# Autodesk Inventor assembly: #Spindexer
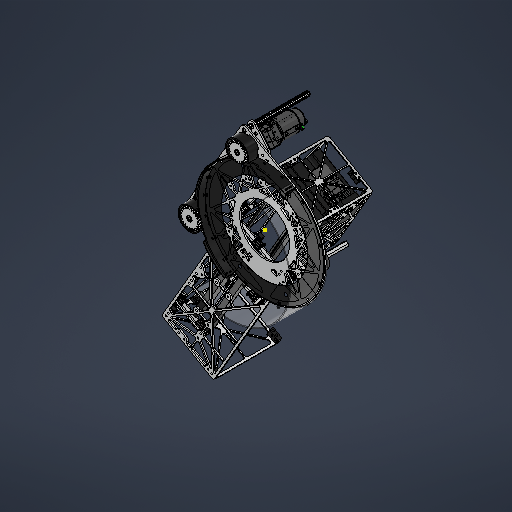
[picture p0: Inventor's stored thumbnail of the model, 512x512]
Saved by Autodesk Inventor 2026.1 (Build 301233020, 233B)
## iProperties
Created: 2026-02-05
Part Number: #Spindexer
Document SubType Name: Assembly
Designer: Owen L
Mass: 5573.01 g
Surface Area: 15044.5 cm^2
Volume: 3852.19 cm^3
Density: 1.44671 g/cm^3
Author: Owen L
## Documents named in this file (58)
- C:\Users\Owen\Documents\GitHub\2026-Robot-Mechanical\Spindexer\#Spindexer.iam
- C:\Users\Owen\Documents\GitHub\2026-Robot-Mechanical\Spindexer\3DPRINT,KICKER,RAMP.ipt
- C:\Users\Owen\Documents\GitHub\2026-Robot-Mechanical\#1_CAD Library\Power Transmission\Bearings\PURCHASED,HEX_BEARING.ipt
- C:\Users\Owen\Documents\GitHub\2026-Robot-Mechanical\#1_CAD Library\Building Materials\Fasteners\Nuts\PURCHASED,NYLOCK,10-32,NUT.ipt
- C:\Users\Owen\Documents\GitHub\2026-Robot-Mechanical\#1_CAD Library\Building Materials\Fasteners\Bolts\PURCHASED,10-32x0.625in,BUTTONHEAD,BOLT.ipt
- C:\Users\Owen\Documents\GitHub\2026-Robot-Mechanical\Spindexer\PLATE,SHOOTER,MOUNT.ipt
- C:\Users\Owen\Documents\GitHub\2026-Robot-Mechanical\Spindexer\PLATE,TURRET,ENCODER,GEAR.ipt
- C:\Users\Owen\Documents\GitHub\2026-Robot-Mechanical\Spindexer\PLATE,TURRET,PINNION,GEAR.ipt
- C:\Users\Owen\Documents\GitHub\2026-Robot-Mechanical\Spindexer\PLATE,TURRET,MOTOR,MOUNT.ipt
- C:\Users\Owen\Documents\GitHub\2026-Robot-Mechanical\#1_CAD Library\Electronics\CONTROLS,ENCODER,HEX_BORE.ipt
- C:\Users\Owen\Documents\GitHub\2026-Robot-Mechanical\Spindexer\STOCK,HEX,SHAFT,TURRET,DRIVE.ipt
- C:\Users\Owen\Documents\GitHub\2026-Robot-Mechanical\Spindexer\STOCK,HEX,SHAFT,TURRET,ENCODER.ipt
- C:\Users\Owen\Documents\GitHub\2026-Robot-Mechanical\Spindexer\3DPRINT,TURRET,HEX,SPACER.ipt
- C:\Users\Owen\Documents\GitHub\2026-Robot-Mechanical\Spindexer\STOCK,CHURRO,HEX,TURRET,MOTOR-MOUNT,SPACER.ipt
- C:\Users\Owen\Documents\GitHub\2026-Robot-Mechanical\#1_CAD Library\Building Materials\Fasteners\Bolts\PURCHASED,0.25-20x0.5in,BUTTONHEAD,BOLT.ipt
- C:\Users\Owen\Documents\GitHub\2026-Robot-Mechanical\Spindexer\MOTOR,VEX,FALCON,500.ipt
- C:\Users\Owen\Documents\GitHub\2026-Robot-Mechanical\#1_CAD Library\Power Transmission\MaxPlanetary\PURCHASED,REV,MAX-PLANETARY,SINGLE-STAGE,FALCON-TO-HEX.ipt
- C:\Users\Owen\Documents\GitHub\2026-Robot-Mechanical\#1_CAD Library\Building Materials\Fasteners\Washers\PURCHASED,WASHER,10-32.ipt
- C:\Users\Owen\Documents\GitHub\2026-Robot-Mechanical\Spindexer\3DPRINT,CABLE-SHROUD,QUARTER.ipt
- C:\Users\Owen\Documents\GitHub\2026-Robot-Mechanical\Spindexer\3DPRINT,CABLE,TRAY,BL.ipt
- C:\Users\Owen\Documents\GitHub\2026-Robot-Mechanical\Spindexer\3DPRINT,CABLE,TRAY,BR.ipt
- C:\Users\Owen\Documents\GitHub\2026-Robot-Mechanical\Spindexer\3DPRINT,CABLE,TRAY,TL.ipt
- C:\Users\Owen\Documents\GitHub\2026-Robot-Mechanical\Spindexer\3DPRINT,CABLE,TRAY,TR.ipt
- C:\Users\Owen\Documents\GitHub\2026-Robot-Mechanical\Spindexer\PLATE,SHOOTER,SHEILD,LOWER.ipt
- C:\Users\Owen\Documents\GitHub\2026-Robot-Mechanical\Spindexer\3DPRINT,TURRET,PINION,SHROUD.ipt
- C:\Users\Owen\Documents\GitHub\2026-Robot-Mechanical\#1_CAD Library\Building Materials\Fasteners\Bolts\PURCHASED,10-32x0.75in,BUTTONHEAD,BOLT.ipt
- C:\Users\Owen\Documents\GitHub\2026-Robot-Mechanical\Spindexer\3DPRINT,TURRET,PINION,SHROUD,21T.ipt
- C:\Users\Owen\Documents\GitHub\2026-Robot-Mechanical\Spindexer\STOCK,CHURRO,HEX,TURRET,MOTOR-MOUNT,SUPPORT.ipt
- C:\Users\Owen\Documents\GitHub\2026-Robot-Mechanical\Spindexer\PLATE,BACK.ipt
- C:\Users\Owen\Documents\GitHub\2026-Robot-Mechanical\Spindexer\PLATE,FRONT.ipt
- C:\Users\Owen\Documents\GitHub\2026-Robot-Mechanical\#1_CAD Library\Wheels\Compliant\PURCHASED,WHEEL,COMPLIANT,2.25in.ipt
- C:\Users\Owen\Documents\GitHub\2026-Robot-Mechanical\Spindexer\PLATE,BEARING,BLOCK.ipt
- C:\Users\Owen\Documents\GitHub\2026-Robot-Mechanical\Spindexer\PLATE,BEARING,BLOCK,TOP.ipt
- C:\Users\Owen\Documents\GitHub\2026-Robot-Mechanical\Spindexer\Kicker.ipt
- C:\Users\Owen\Documents\GitHub\2026-Robot-Mechanical\#1_CAD Library\Motors\MOTOR,NEO,V2.0.ipt
- C:\Users\Owen\Documents\GitHub\2026-Robot-Mechanical\Spindexer\PLATE_LEFT.ipt
- C:\Users\Owen\Documents\GitHub\2026-Robot-Mechanical\Spindexer\PLATE,BELT,REVERSER.ipt
- C:\Users\Owen\Documents\GitHub\2026-Robot-Mechanical\Spindexer\WCP-0562.ipt
- C:\Users\Owen\Documents\GitHub\2026-Robot-Mechanical\Spindexer\REV-21-1921.ipt
- C:\Users\Owen\Documents\GitHub\2026-Robot-Mechanical\Spindexer\WCP-2057.ipt
- C:\Users\Owen\Documents\GitHub\2026-Robot-Mechanical\Spindexer\WCP-1420.ipt
- C:\Users\Owen\Documents\GitHub\2026-Robot-Mechanical\Spindexer\STOCK,LEFT,HEX.ipt
- C:\Users\Owen\Documents\GitHub\2026-Robot-Mechanical\Spindexer\STOCK,REVERSER,HEX.ipt
- C:\Users\Owen\Documents\GitHub\2026-Robot-Mechanical\Spindexer\STOCK,TOP-RIGHT,HEX.ipt
- C:\Users\Owen\Documents\GitHub\2026-Robot-Mechanical\Spindexer\STOCK,BOTTOM-RIGHT,HEX.ipt
- C:\Users\Owen\Documents\GitHub\2026-Robot-Mechanical\Spindexer\3DPRINT,ROLLER,PLUG,SHORT.ipt
- C:\Users\Owen\Documents\GitHub\2026-Robot-Mechanical\Spindexer\3DPRINT,ROLLER,PLUG,LONG.ipt
- C:\Users\Owen\Documents\GitHub\2026-Robot-Mechanical\Spindexer\STOCK,KICKER,HEX.ipt
- C:\Users\Owen\Documents\GitHub\2026-Robot-Mechanical\Spindexer\3DPRINT,VERTICAL,ROLLER,TOP,BEARING,BLOCK.ipt
- C:\Users\Owen\Documents\GitHub\2026-Robot-Mechanical\Spindexer\WCP-0565.ipt
- C:\Users\Owen\Documents\GitHub\2026-Robot-Mechanical\Spindexer\3DPRINT,KICKER,MOTOR,MOUNT.ipt
- C:\Users\Owen\Documents\GitHub\2026-Robot-Mechanical\Spindexer\3DPRINT,NUT-BLOCK.ipt
- C:\Users\Owen\Documents\GitHub\2026-Robot-Mechanical\Spindexer\STOCK,REVERSER,STANDOFF.ipt
- C:\Users\Owen\Documents\GitHub\2026-Robot-Mechanical\Spindexer\3DPRINT,BELT,GUARD.ipt
- C:\Users\Owen\Documents\GitHub\2026-Robot-Mechanical\Spindexer\3DPRINT,BACK,RAIL.ipt
- C:\Users\Owen\Documents\GitHub\2026-Robot-Mechanical\Spindexer\PLATE,RIGHT.ipt
- C:\Users\Owen\Documents\GitHub\2026-Robot-Mechanical\Spindexer\STOCK,VERTICAL,HEX.ipt
- C:\Users\Owen\Documents\GitHub\2026-Robot-Mechanical\Spindexer\3DPRINT,LEFT,NUT-BLOCK.ipt
## Components (152 placed, 57 different names)
1. 3DPRINT,VERTICAL,ROLLER,TOP,BEARING,BLOCK:1 — Mate:309, Insert:317, Mate:359, Mate:360
2. 3DPRINT,TURRET,PINION,SHROUD:1 — Mate:224, Mate:225, Mate:226, Insert:267
3. PURCHASED,10-32x0.75in,BUTTONHEAD,BOLT:1 — Insert:268, Mate:232
4. PURCHASED,10-32x0.75in,BUTTONHEAD,BOLT:2 — Insert:267, Mate:236
5. 3DPRINT,TURRET,PINION,SHROUD,21T:1 — Mate:227, Mate:228, Mate:229, Insert:268
6. STOCK,CHURRO,HEX,TURRET,MOTOR-MOUNT,SPACER:7 — Insert:272
7. STOCK,CHURRO,HEX,TURRET,MOTOR-MOUNT,SPACER:8 — Insert:273
8. PURCHASED,0.25-20x0.5in,BUTTONHEAD,BOLT:16 — Insert:279
9. PURCHASED,0.25-20x0.5in,BUTTONHEAD,BOLT:17 — Insert:280
10. PURCHASED,0.25-20x0.5in,BUTTONHEAD,BOLT:18 — Insert:281
11. STOCK,CHURRO,HEX,TURRET,MOTOR-MOUNT,SUPPORT:1 — Insert:282
12. PLATE,BACK:1 — Mate:240, Mate:264, Flush:44, Flush:48, Flush:52, Mate:277, Mate:278, Mate:280, Insert:305, Insert:306, Insert:309, Insert:312, Insert:314, Insert:316, Mate:269, Insert:318, Mate:314, Mate:315, Insert:322, Insert:323, Mate:331, Mate:332, Insert:324, Insert:325, Mate:333, Mate:334, Mate:336, Mate:337, Mate:338, Insert:328, Insert:333, Insert:334, Insert:335, Insert:336, Insert:337, Insert:338, Mate:344, Insert:339, Mate:347, Flush:71, Mate:351, Flush:73, Mate:352, Flush:74, Flush:75, Mate:357, Flush:76, Insert:342, Mate:362
13. PLATE,FRONT:1 — Mate:264, Flush:44, Mate:265, Mate:268, Mate:270, Mate:274, Flush:51, Insert:311, Insert:313, Insert:315, Mate:306, Mate:311, Mate:323, Insert:320, Mate:325, Mate:327, Mate:328, Mate:329, Insert:326, Mate:335, Insert:327, Insert:331, Insert:332, Mate:339, Mate:340, Mate:343, Mate:345, Insert:340
14. PURCHASED,WHEEL,COMPLIANT,2.25in:1 — Mate:268, Mate:269, Insert:298, Mate:270
15. PURCHASED,WHEEL,COMPLIANT,2.25in:3 — Insert:298, Mate:309
16. PLATE,BEARING,BLOCK:1 — Flush:48, Flush:53, Insert:308
17. PLATE,BEARING,BLOCK,TOP:1 — Mate:272, Mate:278, Flush:53, Insert:310
18. KICKER_GEARBOX — Insert:304, Flush:50, Mate:323, Mate:325, Mate:326
19. MOTOR,NEO,V2.0:1 — Insert:304, Flush:50
20. PLATE,LEFT — Mate:274, Flush:51, Mate:275, Insert:341, Mate:353, Mate:354, Mate:355, Mate:356
21. PLATE,BELT,REVERSER:1 — Mate:280, Insert:307
22. WCP-0562:1 — Mate:285, Flush:56, Flush:58
23. REV-21-1921:1 — Mate:282, Flush:54
24. REV-21-1921:2 — Mate:281, Flush:54, Mate:290, Mate:291
25. WCP-2057:1 — Insert:308, Mate:287, Flush:59
26. WCP-2057:2 — Insert:307, Mate:283, Mate:291, Flush:60
27. WCP-2057:3 — Insert:306, Mate:282, Mate:287, Mate:292, Mate:296
28. WCP-2057:4 — Insert:305, Mate:281, Mate:288, Mate:289, Mate:297
29. WCP-2057:5 — Insert:311, Flush:62
30. WCP-2057:6 — Insert:310, Mate:286, Flush:61
31. WCP-2057:7 — Insert:313, Flush:63
32. WCP-2057:8 — Insert:309, Mate:284, Mate:285, Mate:286, Mate:295
33. WCP-2057:9 — Insert:312, Mate:293, Mate:299, Mate:316, Mate:318
34. WCP-2057:11 — Insert:314, Mate:294, Mate:300
35. WCP-2057:12 — Insert:316, Mate:319
36. WCP-2057:13 — Insert:315, Mate:301, Mate:302, Mate:305, Mate:324
37. WCP-1420:1 — Mate:283, Mate:288, Flush:55, Mate:289, Mate:290
38. WCP-1420:2 — Mate:284, Flush:55
39. WCP-0562:2 — Mate:292, Flush:56
40. WCP-0562:3 — Mate:293, Flush:57, Flush:58
41. WCP-0562:4 — Mate:294, Flush:57
42. STOCK,LEFT,HEX:1 — Mate:295, Flush:61
43. STOCK,LEFT,HEX:2 — Mate:296, Flush:59
44. STOCK,REVERSER,HEX:1 — Mate:297, Flush:60
45. STOCK,TOP-RIGHT,HEX:1 — Mate:299, Flush:62
46. STOCK,BOTTOM-RIGHT,HEX:1 — Mate:300, Flush:63
47. 3DPRINT,ROLLER,PLUG,SHORT:1
48. 3DPRINT,ROLLER,PLUG,LONG:1
49. STOCK,KICKER,HEX:1 — Mate:301
50. WCP-1420:3 — Mate:302, Flush:65, Mate:324
51. WCP-1420:5 — Mate:305, Mate:311
52. WCP-1420:6 — Mate:359, Mate:360, Flush:77
53. WCP-1420:7 — Mate:306, Flush:65, Mate:326
54. WCP-2057:14 — Insert:317, Mate:361
55. PLATE,BELT,REVERSER:2 — Mate:314, Mate:315, Insert:319
56. REV-21-1921:3 — Mate:317, Flush:66, Mate:321
57. WCP-2057:15 — Insert:318, Mate:317, Mate:320
58. REV-21-1921:4 — Mate:316, Mate:318, Flush:66
59. WCP-0565:1 — Mate:319, Flush:67
60. WCP-1420:8 — Mate:320, Mate:321, Mate:322, Flush:67
61. WCP-2057:16 — Insert:319, Mate:322
62. WCP-2057:17 — Insert:320
63. 3DPRINT,KICKER,MOTOR,MOUNT:1 — Mate:327, Mate:328, Mate:329
64. 3DPRINT,NUT-BLOCK:1 — Insert:321, Mate:330
65. 3DPRINT,NUT-BLOCK:2 — Insert:323, Mate:332
66. 3DPRINT,NUT-BLOCK:3 — Insert:322, Mate:331
67. 3DPRINT,NUT-BLOCK:4 — Insert:324, Mate:333
68. 3DPRINT,NUT-BLOCK:5 — Insert:325, Mate:334
69. 3DPRINT,NUT-BLOCK:6 — Insert:326, Mate:335
70. 3DPRINT,NUT-BLOCK:7 — Mate:336, Mate:337, Mate:338
71. 3DPRINT,NUT-BLOCK:8 — Insert:327, Mate:343
72. 3DPRINT,NUT-BLOCK:9 — Insert:332, Mate:339
73. 3DPRINT,NUT-BLOCK:10 — Insert:331, Mate:340
74. 3DPRINT,NUT-BLOCK:11 — Mate:345, Insert:340
75. 3DPRINT,NUT-BLOCK:12 — Mate:344, Insert:339
76. 3DPRINT,NUT-BLOCK:13 — Insert:328
77. STOCK,REVERSER,STANDOFF:1 — Insert:333
78. STOCK,REVERSER,STANDOFF:2 — Insert:334
79. STOCK,REVERSER,STANDOFF:3 — Insert:335
80. STOCK,REVERSER,STANDOFF:4 — Insert:338
81. STOCK,REVERSER,STANDOFF:5 — Insert:337
82. STOCK,REVERSER,STANDOFF:6 — Insert:336
83. 3DPRINT,BELT,GUARD:1 — Mate:346, Mate:347, Mate:348, Flush:68, Flush:72
84. 3DPRINT,BELT,GUARD:2 — Mate:348, Mate:349, Flush:68
85. 3DPRINT,BELT,GUARD:3 — Flush:70, Flush:71, Mate:351, Flush:72
86. 3DPRINT,BELT,GUARD:4 — Flush:70, Flush:73
87. 3DPRINT,BACK,RAIL:1 — Mate:352, Flush:74, Flush:75
88. 3DPRINT,NUT-BLOCK:14 — Insert:341, Mate:353
89. 3DPRINT,NUT-BLOCK:15 — Mate:354, Mate:355, Mate:356
90. PLATE,RIGHT:1 — Mate:357, Mate:358, Flush:76, Mate:364, Insert:344
91. STOCK,VERTICAL,HEX:1 — Mate:361, Flush:77
92. 3DPRINT,NUT-BLOCK:16 — Insert:343, Mate:363
93. 3DPRINT,NUT-BLOCK:17 — Insert:342, Mate:362
94. 3DPRINT,LEFT,NUT-BLOCK:1 — Mate:364, Insert:344
95. PURCHASED,10-32x0.625in,BUTTONHEAD,BOLT:45 — Insert:233
96. PURCHASED,NYLOCK,10-32,NUT:5 — Insert:234
97. PURCHASED,NYLOCK,10-32,NUT:6 — Insert:232
98. PURCHASED,0.25-20x0.5in,BUTTONHEAD,BOLT:9 — Insert:163
99. PURCHASED,0.25-20x0.5in,BUTTONHEAD,BOLT:8 — Insert:162
100. PURCHASED,0.25-20x0.5in,BUTTONHEAD,BOLT:6 — Insert:159
101. PURCHASED,0.25-20x0.5in,BUTTONHEAD,BOLT:5 — Insert:270
102. PURCHASED,NYLOCK,10-32,NUT:8 — Insert:236
103. PURCHASED,NYLOCK,10-32,NUT:7 — Insert:238
104. PURCHASED,10-32x0.625in,BUTTONHEAD,BOLT:47 — Insert:235
105. PURCHASED,0.25-20x0.5in,BUTTONHEAD,BOLT:4 — Insert:158
106. PURCHASED,10-32x0.625in,BUTTONHEAD,BOLT:61 — Insert:174
107. PURCHASED,10-32x0.625in,BUTTONHEAD,BOLT:60 — Insert:175
108. PURCHASED,10-32x0.625in,BUTTONHEAD,BOLT:59 — Insert:176
109. PURCHASED,10-32x0.625in,BUTTONHEAD,BOLT:58 — Insert:177
110. PURCHASED,0.25-20x0.5in,BUTTONHEAD,BOLT:15 — Insert:277
111. PURCHASED,0.25-20x0.5in,BUTTONHEAD,BOLT:14 — Insert:278
112. PURCHASED,0.25-20x0.5in,BUTTONHEAD,BOLT:13
113. PURCHASED,0.25-20x0.5in,BUTTONHEAD,BOLT:12 — Insert:276
114. PURCHASED,0.25-20x0.5in,BUTTONHEAD,BOLT:11 — Insert:169
115. PURCHASED,0.25-20x0.5in,BUTTONHEAD,BOLT:10 — Insert:168
116. PURCHASED,WASHER,10-32:11 — Insert:215, Insert:218
117. PURCHASED,WASHER,10-32:12 — Insert:217, Insert:220
118. PURCHASED,WASHER,10-32:13 — Insert:216, Insert:219
119. PURCHASED,10-32x0.625in,BUTTONHEAD,BOLT:62 — Insert:218
120. PURCHASED,10-32x0.625in,BUTTONHEAD,BOLT:63 — Insert:219
121. PURCHASED,10-32x0.625in,BUTTONHEAD,BOLT:64 — Insert:220
122. 3DPRINT,TURRET,HEX,SPACER:1 — Mate:94, Mate:102, Mate:144, Mate:145
123. 3DPRINT,TURRET,HEX,SPACER:2 — Mate:93, Mate:141, Mate:142
124. 3DPRINT,KICKER,RAMP:1 — Flush:52, Mate:277
125. 3DPRINT,CABLE,TRAY,TR:1 — Mate:219, Mate:220
126. 3DPRINT,CABLE,TRAY,TL:1 — Mate:217, Mate:218, Mate:219, Mate:220
127. 3DPRINT,CABLE,TRAY,BR:1 — Mate:215, Mate:216, Mate:217, Mate:218
128. 3DPRINT,CABLE,TRAY,BL:1 — Mate:213, Mate:214, Flush:33, Mate:215, Mate:216
129. 3DPRINT,CABLE-SHROUD,QUARTER:2 — Mate:205, Mate:206, Mate:207, Mate:223, Mate:226
130. 3DPRINT,CABLE-SHROUD,QUARTER:1 — Mate:202, Mate:203, Mate:204, Mate:205, Mate:207, Flush:33, Mate:228
131. PLATE,SHOOTER,MOUNT:1 — Mate:82, Mate:95, Mate:100, Insert:150, Insert:152, Insert:153, Insert:154, Insert:158, Insert:159, Insert:165, Insert:166, Insert:168, Insert:169, Insert:233, Insert:235, Mate:202, Mate:203, Mate:204, Mate:206, Mate:213, Mate:214, Mate:222, Flush:34, Mate:225, Mate:229, Mate:231, Insert:270, Mate:233, Mate:234, Mate:235, Insert:274, Insert:276, Insert:280, Insert:281, Mate:240, Mate:265, Mate:272, Mate:275, Insert:321, Mate:330, Mate:346, Mate:349, Mate:358, Insert:343, Mate:363
132. PLATE,TURRET,MOTOR,MOUNT:1 — Mate:100, Insert:155, Insert:157, Insert:162, Insert:163, Insert:174, Insert:175, Insert:176, Insert:177, Mate:147, Insert:178, Mate:148, Mate:231, Insert:269, Insert:282
133. PLATE,TURRET,MOTOR,MOUNT:2 — Mate:233, Mate:234, Mate:235, Insert:271, Insert:272, Insert:273, Insert:275, Insert:277, Insert:278, Insert:279
134. PLATE,TURRET,ENCODER,GEAR:1 — Mate:102, Mate:143, Flush:26
135. PLATE,TURRET,PINNION,GEAR:1 — Mate:86, Flush:25, Mate:140, Mate:141
136. PLATE,SHOOTER,SHEILD,LOWER:1 — Mate:222, Flush:34, Mate:223
137. STOCK,CHURRO,HEX,TURRET,MOTOR-MOUNT,SPACER:5 — Insert:165
138. STOCK,CHURRO,HEX,TURRET,MOTOR-MOUNT,SPACER:6 — Insert:166
139. STOCK,CHURRO,HEX,TURRET,MOTOR-MOUNT,SPACER:4 — Insert:271, Insert:274
140. STOCK,CHURRO,HEX,TURRET,MOTOR-MOUNT,SPACER:3 — Insert:269
141. STOCK,CHURRO,HEX,TURRET,MOTOR-MOUNT,SPACER:2 — Insert:152, Insert:157
142. STOCK,CHURRO,HEX,TURRET,MOTOR-MOUNT,SPACER:1 — Insert:150
143. STOCK,HEX,SHAFT,TURRET,ENCODER:1 — Mate:143, Flush:26, Mate:144, Insert:216, Insert:217, Mate:224
144. STOCK,HEX,SHAFT,TURRET,DRIVE:1 — Flush:25, Mate:140, Mate:142, Insert:215, Mate:227
145. PURCHASED,HEX_BEARING:6 — Mate:83, Mate:86, Mate:93, Insert:154
146. PURCHASED,HEX_BEARING:7 — Mate:94, Mate:96, Insert:153, Mate:145
147. CONTROLS,ENCODER,HEX_BORE:1 — Mate:95, Mate:96, Insert:236, Insert:238, Mate:236
148. CONTROLS,ENCODER,HEX_BORE:2 — Mate:82, Mate:83, Insert:232, Insert:234, Mate:232
149. PURCHASED,HEX_BEARING:8 — Insert:155
150. MOTOR,VEX,FALCON,500:1 — Insert:179, Mate:149
151. PURCHASED,REV,MAX-PLANETARY,SINGLE-STAGE,FALCON-TO-HEX:1 — Mate:147, Insert:178, Mate:148, Insert:179, Mate:149
152. PURCHASED,HEX_BEARING:9 — Insert:275
## Relationships (256: Mate 135, Insert 88, Flush 33)
- Mate:82: PLATE,SHOOTER,MOUNT:1 ↔ CONTROLS,ENCODER,HEX_BORE:2
- Mate:83: PURCHASED,HEX_BEARING:6 ↔ CONTROLS,ENCODER,HEX_BORE:2
- Mate:86: PLATE,TURRET,PINNION,GEAR:1 ↔ PURCHASED,HEX_BEARING:6
- Mate:93: 3DPRINT,TURRET,HEX,SPACER:2 ↔ PURCHASED,HEX_BEARING:6
- Mate:94: 3DPRINT,TURRET,HEX,SPACER:1 ↔ PURCHASED,HEX_BEARING:7
- Mate:95: PLATE,SHOOTER,MOUNT:1 ↔ CONTROLS,ENCODER,HEX_BORE:1
- Mate:96: PURCHASED,HEX_BEARING:7 ↔ CONTROLS,ENCODER,HEX_BORE:1
- Mate:100 (19.05 mm): PLATE,SHOOTER,MOUNT:1 ↔ PLATE,TURRET,MOTOR,MOUNT:1
- Mate:102: 3DPRINT,TURRET,HEX,SPACER:1 ↔ PLATE,TURRET,ENCODER,GEAR:1
- Insert:150: PLATE,SHOOTER,MOUNT:1 ↔ STOCK,CHURRO,HEX,TURRET,MOTOR-MOUNT,SPACER:1
- Insert:152: PLATE,SHOOTER,MOUNT:1 ↔ STOCK,CHURRO,HEX,TURRET,MOTOR-MOUNT,SPACER:2
- Insert:153: PLATE,SHOOTER,MOUNT:1 ↔ PURCHASED,HEX_BEARING:7
- Insert:154: PLATE,SHOOTER,MOUNT:1 ↔ PURCHASED,HEX_BEARING:6
- Insert:155: PLATE,TURRET,MOTOR,MOUNT:1 ↔ PURCHASED,HEX_BEARING:8
- Insert:157: PLATE,TURRET,MOTOR,MOUNT:1 ↔ STOCK,CHURRO,HEX,TURRET,MOTOR-MOUNT,SPACER:2
- Insert:158: PURCHASED,0.25-20x0.5in,BUTTONHEAD,BOLT:4 ↔ PLATE,SHOOTER,MOUNT:1
- Insert:159: PURCHASED,0.25-20x0.5in,BUTTONHEAD,BOLT:6 ↔ PLATE,SHOOTER,MOUNT:1
- Insert:162: PURCHASED,0.25-20x0.5in,BUTTONHEAD,BOLT:8 ↔ PLATE,TURRET,MOTOR,MOUNT:1
- Insert:163: PURCHASED,0.25-20x0.5in,BUTTONHEAD,BOLT:9 ↔ PLATE,TURRET,MOTOR,MOUNT:1
- Flush:25: PLATE,TURRET,PINNION,GEAR:1 ↔ STOCK,HEX,SHAFT,TURRET,DRIVE:1
- Mate:140: PLATE,TURRET,PINNION,GEAR:1 ↔ STOCK,HEX,SHAFT,TURRET,DRIVE:1
- Mate:141: 3DPRINT,TURRET,HEX,SPACER:2 ↔ PLATE,TURRET,PINNION,GEAR:1
- Mate:142: 3DPRINT,TURRET,HEX,SPACER:2 ↔ STOCK,HEX,SHAFT,TURRET,DRIVE:1
- Mate:143: PLATE,TURRET,ENCODER,GEAR:1 ↔ STOCK,HEX,SHAFT,TURRET,ENCODER:1
- Flush:26: PLATE,TURRET,ENCODER,GEAR:1 ↔ STOCK,HEX,SHAFT,TURRET,ENCODER:1
- Mate:144: 3DPRINT,TURRET,HEX,SPACER:1 ↔ STOCK,HEX,SHAFT,TURRET,ENCODER:1
- Mate:145: 3DPRINT,TURRET,HEX,SPACER:1 ↔ PURCHASED,HEX_BEARING:7
- Insert:165: PLATE,SHOOTER,MOUNT:1 ↔ STOCK,CHURRO,HEX,TURRET,MOTOR-MOUNT,SPACER:5
- Insert:166: PLATE,SHOOTER,MOUNT:1 ↔ STOCK,CHURRO,HEX,TURRET,MOTOR-MOUNT,SPACER:6
- Insert:168: PURCHASED,0.25-20x0.5in,BUTTONHEAD,BOLT:10 ↔ PLATE,SHOOTER,MOUNT:1
- Insert:169: PURCHASED,0.25-20x0.5in,BUTTONHEAD,BOLT:11 ↔ PLATE,SHOOTER,MOUNT:1
- Insert:174: PURCHASED,10-32x0.625in,BUTTONHEAD,BOLT:61 ↔ PLATE,TURRET,MOTOR,MOUNT:1
- Insert:175: PURCHASED,10-32x0.625in,BUTTONHEAD,BOLT:60 ↔ PLATE,TURRET,MOTOR,MOUNT:1
- Insert:176: PURCHASED,10-32x0.625in,BUTTONHEAD,BOLT:59 ↔ PLATE,TURRET,MOTOR,MOUNT:1
- Insert:177: PURCHASED,10-32x0.625in,BUTTONHEAD,BOLT:58 ↔ PLATE,TURRET,MOTOR,MOUNT:1
- Mate:147: PLATE,TURRET,MOTOR,MOUNT:1 ↔ PURCHASED,REV,MAX-PLANETARY,SINGLE-STAGE,FALCON-TO-HEX:1
- Insert:178: PLATE,TURRET,MOTOR,MOUNT:1 ↔ PURCHASED,REV,MAX-PLANETARY,SINGLE-STAGE,FALCON-TO-HEX:1
- Mate:148: PLATE,TURRET,MOTOR,MOUNT:1 ↔ PURCHASED,REV,MAX-PLANETARY,SINGLE-STAGE,FALCON-TO-HEX:1
- Insert:179: MOTOR,VEX,FALCON,500:1 ↔ PURCHASED,REV,MAX-PLANETARY,SINGLE-STAGE,FALCON-TO-HEX:1
- Mate:149: MOTOR,VEX,FALCON,500:1 ↔ PURCHASED,REV,MAX-PLANETARY,SINGLE-STAGE,FALCON-TO-HEX:1
- Insert:215: PURCHASED,WASHER,10-32:11 ↔ STOCK,HEX,SHAFT,TURRET,DRIVE:1
- Insert:216: PURCHASED,WASHER,10-32:13 ↔ STOCK,HEX,SHAFT,TURRET,ENCODER:1
- Insert:217: PURCHASED,WASHER,10-32:12 ↔ STOCK,HEX,SHAFT,TURRET,ENCODER:1
- Insert:218: PURCHASED,WASHER,10-32:11 ↔ PURCHASED,10-32x0.625in,BUTTONHEAD,BOLT:62
- Insert:219: PURCHASED,WASHER,10-32:13 ↔ PURCHASED,10-32x0.625in,BUTTONHEAD,BOLT:63
- Insert:220: PURCHASED,WASHER,10-32:12 ↔ PURCHASED,10-32x0.625in,BUTTONHEAD,BOLT:64
- Insert:232: PURCHASED,NYLOCK,10-32,NUT:6 ↔ CONTROLS,ENCODER,HEX_BORE:2
- Insert:233: PURCHASED,10-32x0.625in,BUTTONHEAD,BOLT:45 ↔ PLATE,SHOOTER,MOUNT:1
- Insert:234: PURCHASED,NYLOCK,10-32,NUT:5 ↔ CONTROLS,ENCODER,HEX_BORE:2
- Insert:235: PURCHASED,10-32x0.625in,BUTTONHEAD,BOLT:47 ↔ PLATE,SHOOTER,MOUNT:1
- Insert:236: PURCHASED,NYLOCK,10-32,NUT:8 ↔ CONTROLS,ENCODER,HEX_BORE:1
- Insert:238: PURCHASED,NYLOCK,10-32,NUT:7 ↔ CONTROLS,ENCODER,HEX_BORE:1
- Mate:202: 3DPRINT,CABLE-SHROUD,QUARTER:1 ↔ PLATE,SHOOTER,MOUNT:1
- Mate:203: 3DPRINT,CABLE-SHROUD,QUARTER:1 ↔ PLATE,SHOOTER,MOUNT:1
- Mate:204: 3DPRINT,CABLE-SHROUD,QUARTER:1 ↔ PLATE,SHOOTER,MOUNT:1
- Mate:205: 3DPRINT,CABLE-SHROUD,QUARTER:2 ↔ 3DPRINT,CABLE-SHROUD,QUARTER:1
- Mate:206: 3DPRINT,CABLE-SHROUD,QUARTER:2 ↔ PLATE,SHOOTER,MOUNT:1
- Mate:207: 3DPRINT,CABLE-SHROUD,QUARTER:2 ↔ 3DPRINT,CABLE-SHROUD,QUARTER:1
- Mate:213: 3DPRINT,CABLE,TRAY,BL:1 ↔ PLATE,SHOOTER,MOUNT:1
- Mate:214: 3DPRINT,CABLE,TRAY,BL:1 ↔ PLATE,SHOOTER,MOUNT:1
- Flush:33: 3DPRINT,CABLE,TRAY,BL:1 ↔ 3DPRINT,CABLE-SHROUD,QUARTER:1
- Mate:215: 3DPRINT,CABLE,TRAY,BR:1 ↔ 3DPRINT,CABLE,TRAY,BL:1
- Mate:216: 3DPRINT,CABLE,TRAY,BR:1 ↔ 3DPRINT,CABLE,TRAY,BL:1
- Mate:217: 3DPRINT,CABLE,TRAY,TL:1 ↔ 3DPRINT,CABLE,TRAY,BR:1
- Mate:218: 3DPRINT,CABLE,TRAY,TL:1 ↔ 3DPRINT,CABLE,TRAY,BR:1
- Mate:219: 3DPRINT,CABLE,TRAY,TR:1 ↔ 3DPRINT,CABLE,TRAY,TL:1
- Mate:220: 3DPRINT,CABLE,TRAY,TR:1 ↔ 3DPRINT,CABLE,TRAY,TL:1
- Mate:222: PLATE,SHOOTER,MOUNT:1 ↔ PLATE,SHOOTER,SHEILD,LOWER:1
- Flush:34: PLATE,SHOOTER,MOUNT:1 ↔ PLATE,SHOOTER,SHEILD,LOWER:1
- Mate:223: 3DPRINT,CABLE-SHROUD,QUARTER:2 ↔ PLATE,SHOOTER,SHEILD,LOWER:1
- Mate:224: 3DPRINT,TURRET,PINION,SHROUD:1 ↔ STOCK,HEX,SHAFT,TURRET,ENCODER:1
- Mate:225: 3DPRINT,TURRET,PINION,SHROUD:1 ↔ PLATE,SHOOTER,MOUNT:1
- Mate:226: 3DPRINT,TURRET,PINION,SHROUD:1 ↔ 3DPRINT,CABLE-SHROUD,QUARTER:2
- Insert:267: 3DPRINT,TURRET,PINION,SHROUD:1 ↔ PURCHASED,10-32x0.75in,BUTTONHEAD,BOLT:2
- Mate:227: 3DPRINT,TURRET,PINION,SHROUD,21T:1 ↔ STOCK,HEX,SHAFT,TURRET,DRIVE:1
- Mate:228: 3DPRINT,TURRET,PINION,SHROUD,21T:1 ↔ 3DPRINT,CABLE-SHROUD,QUARTER:1
- Mate:229: 3DPRINT,TURRET,PINION,SHROUD,21T:1 ↔ PLATE,SHOOTER,MOUNT:1
- Insert:268: PURCHASED,10-32x0.75in,BUTTONHEAD,BOLT:1 ↔ 3DPRINT,TURRET,PINION,SHROUD,21T:1
- Mate:231: PLATE,SHOOTER,MOUNT:1 ↔ PLATE,TURRET,MOTOR,MOUNT:1
- Insert:269: PLATE,TURRET,MOTOR,MOUNT:1 ↔ STOCK,CHURRO,HEX,TURRET,MOTOR-MOUNT,SPACER:3
- Insert:270: PURCHASED,0.25-20x0.5in,BUTTONHEAD,BOLT:5 ↔ PLATE,SHOOTER,MOUNT:1
- Mate:232: PURCHASED,10-32x0.75in,BUTTONHEAD,BOLT:1 ↔ CONTROLS,ENCODER,HEX_BORE:2
- Mate:233: PLATE,SHOOTER,MOUNT:1 ↔ PLATE,TURRET,MOTOR,MOUNT:2
- Mate:234: PLATE,SHOOTER,MOUNT:1 ↔ PLATE,TURRET,MOTOR,MOUNT:2
- Mate:235: PLATE,SHOOTER,MOUNT:1 ↔ PLATE,TURRET,MOTOR,MOUNT:2
- Insert:271: PLATE,TURRET,MOTOR,MOUNT:2 ↔ STOCK,CHURRO,HEX,TURRET,MOTOR-MOUNT,SPACER:4
- Insert:272: STOCK,CHURRO,HEX,TURRET,MOTOR-MOUNT,SPACER:7 ↔ PLATE,TURRET,MOTOR,MOUNT:2
- Insert:273: STOCK,CHURRO,HEX,TURRET,MOTOR-MOUNT,SPACER:8 ↔ PLATE,TURRET,MOTOR,MOUNT:2
- Insert:274: PLATE,SHOOTER,MOUNT:1 ↔ STOCK,CHURRO,HEX,TURRET,MOTOR-MOUNT,SPACER:4
- Insert:275: PLATE,TURRET,MOTOR,MOUNT:2 ↔ PURCHASED,HEX_BEARING:9
- Insert:276: PURCHASED,0.25-20x0.5in,BUTTONHEAD,BOLT:12 ↔ PLATE,SHOOTER,MOUNT:1
- Insert:277: PURCHASED,0.25-20x0.5in,BUTTONHEAD,BOLT:15 ↔ PLATE,TURRET,MOTOR,MOUNT:2
- Insert:278: PURCHASED,0.25-20x0.5in,BUTTONHEAD,BOLT:14 ↔ PLATE,TURRET,MOTOR,MOUNT:2
- Mate:236: PURCHASED,10-32x0.75in,BUTTONHEAD,BOLT:2 ↔ CONTROLS,ENCODER,HEX_BORE:1
- Insert:279: PURCHASED,0.25-20x0.5in,BUTTONHEAD,BOLT:16 ↔ PLATE,TURRET,MOTOR,MOUNT:2
- Insert:280: PURCHASED,0.25-20x0.5in,BUTTONHEAD,BOLT:17 ↔ PLATE,SHOOTER,MOUNT:1
- Insert:281: PURCHASED,0.25-20x0.5in,BUTTONHEAD,BOLT:18 ↔ PLATE,SHOOTER,MOUNT:1
- Insert:282: STOCK,CHURRO,HEX,TURRET,MOTOR-MOUNT,SUPPORT:1 ↔ PLATE,TURRET,MOTOR,MOUNT:1
- Mate:240: PLATE,BACK:1 ↔ PLATE,SHOOTER,MOUNT:1
- Mate:264 (158.75 mm): PLATE,BACK:1 ↔ PLATE,FRONT:1
- Flush:44: PLATE,BACK:1 ↔ PLATE,FRONT:1
- Mate:265: PLATE,FRONT:1 ↔ PLATE,SHOOTER,MOUNT:1
- Mate:268 (-208.788 mm): PLATE,FRONT:1 ↔ PURCHASED,WHEEL,COMPLIANT,2.25in:1
- Mate:269 (179.832 mm): PLATE,BACK:1 ↔ PURCHASED,WHEEL,COMPLIANT,2.25in:1
- Insert:298: PURCHASED,WHEEL,COMPLIANT,2.25in:1 ↔ PURCHASED,WHEEL,COMPLIANT,2.25in:3
- Mate:270 (6.35 mm): PLATE,FRONT:1 ↔ PURCHASED,WHEEL,COMPLIANT,2.25in:1
- Mate:272: PLATE,BEARING,BLOCK,TOP:1 ↔ PLATE,SHOOTER,MOUNT:1
- Flush:48: PLATE,BACK:1 ↔ PLATE,BEARING,BLOCK:1
- Insert:304: KICKER_GEARBOX ↔ MOTOR,NEO,V2.0:1
- Flush:50: KICKER_GEARBOX ↔ MOTOR,NEO,V2.0:1
- Mate:274: PLATE,FRONT:1 ↔ PLATE,LEFT
- Flush:51: PLATE,FRONT:1 ↔ PLATE,LEFT
- Mate:275: PLATE,LEFT ↔ PLATE,SHOOTER,MOUNT:1
- Flush:52: PLATE,BACK:1 ↔ 3DPRINT,KICKER,RAMP:1
- Mate:277: PLATE,BACK:1 ↔ 3DPRINT,KICKER,RAMP:1
- Mate:278 (95.25 mm): PLATE,BACK:1 ↔ PLATE,BEARING,BLOCK,TOP:1
- Flush:53: PLATE,BEARING,BLOCK:1 ↔ PLATE,BEARING,BLOCK,TOP:1
- Mate:280: PLATE,BACK:1 ↔ PLATE,BELT,REVERSER:1
- Insert:305: PLATE,BACK:1 ↔ WCP-2057:4
- Insert:306: PLATE,BACK:1 ↔ WCP-2057:3
- Insert:307: PLATE,BELT,REVERSER:1 ↔ WCP-2057:2
- Insert:308: PLATE,BEARING,BLOCK:1 ↔ WCP-2057:1
- Insert:309: PLATE,BACK:1 ↔ WCP-2057:8
- Insert:310: PLATE,BEARING,BLOCK,TOP:1 ↔ WCP-2057:6
- Insert:311: PLATE,FRONT:1 ↔ WCP-2057:5
- Insert:312: PLATE,BACK:1 ↔ WCP-2057:9
- Insert:313: PLATE,FRONT:1 ↔ WCP-2057:7
- Insert:314: PLATE,BACK:1 ↔ WCP-2057:11
- Insert:315: PLATE,FRONT:1 ↔ WCP-2057:13
- Insert:316: PLATE,BACK:1 ↔ WCP-2057:12
- Mate:281: REV-21-1921:2 ↔ WCP-2057:4
- Mate:282: REV-21-1921:1 ↔ WCP-2057:3
- Flush:54: REV-21-1921:1 ↔ REV-21-1921:2
- Mate:283: WCP-2057:2 ↔ WCP-1420:1
- Mate:284: WCP-2057:8 ↔ WCP-1420:2
- Mate:285: WCP-0562:1 ↔ WCP-2057:8
- Mate:286: WCP-2057:6 ↔ WCP-2057:8
- Mate:287: WCP-2057:1 ↔ WCP-2057:3
- Mate:288: WCP-2057:4 ↔ WCP-1420:1
- Flush:55: WCP-1420:1 ↔ WCP-1420:2
- Mate:289: WCP-2057:4 ↔ WCP-1420:1
- Mate:290: REV-21-1921:2 ↔ WCP-1420:1
- Mate:291: REV-21-1921:2 ↔ WCP-2057:2
- Mate:292: WCP-2057:3 ↔ WCP-0562:2
- Mate:293: WCP-2057:9 ↔ WCP-0562:3
- Mate:294: WCP-2057:11 ↔ WCP-0562:4
- Flush:56: WCP-0562:1 ↔ WCP-0562:2
- Flush:57: WCP-0562:3 ↔ WCP-0562:4
- Flush:58: WCP-0562:1 ↔ WCP-0562:3
- Mate:295: WCP-2057:8 ↔ STOCK,LEFT,HEX:1
- Mate:296: WCP-2057:3 ↔ STOCK,LEFT,HEX:2
- Mate:297: WCP-2057:4 ↔ STOCK,REVERSER,HEX:1
- Mate:299: WCP-2057:9 ↔ STOCK,TOP-RIGHT,HEX:1
- Mate:300: WCP-2057:11 ↔ STOCK,BOTTOM-RIGHT,HEX:1
- Flush:59: WCP-2057:1 ↔ STOCK,LEFT,HEX:2
- Flush:60: WCP-2057:2 ↔ STOCK,REVERSER,HEX:1
- Flush:61: WCP-2057:6 ↔ STOCK,LEFT,HEX:1
- Flush:62: WCP-2057:5 ↔ STOCK,TOP-RIGHT,HEX:1
- Flush:63: WCP-2057:7 ↔ STOCK,BOTTOM-RIGHT,HEX:1
- Mate:301: WCP-2057:13 ↔ STOCK,KICKER,HEX:1
- Mate:302: WCP-2057:13 ↔ WCP-1420:3
- Mate:305: WCP-2057:13 ↔ WCP-1420:5
- Mate:306: PLATE,FRONT:1 ↔ WCP-1420:7
- [Mate]: 3DPRINT,VERTICAL,ROLLER,TOP,BEARING,BLOCK:1 ↔ PURCHASED,WHEEL,COMPLIANT,2.25in:3
- [Mate]: 3DPRINT,VERTICAL,ROLLER,TOP,BEARING,BLOCK:1 ↔ PLATE,FRONT:1
- Mate:309 (12.7 mm): 3DPRINT,VERTICAL,ROLLER,TOP,BEARING,BLOCK:1 ↔ PURCHASED,WHEEL,COMPLIANT,2.25in:3
- Insert:317: 3DPRINT,VERTICAL,ROLLER,TOP,BEARING,BLOCK:1 ↔ WCP-2057:14
- Flush:65: WCP-1420:3 ↔ WCP-1420:7
- Mate:311 (10.7632 mm): PLATE,FRONT:1 ↔ WCP-1420:5
- [Mate]: REV-21-1921:3 ↔ WCP-2057:15
- Insert:318: PLATE,BACK:1 ↔ WCP-2057:15
- Mate:314: PLATE,BACK:1 ↔ PLATE,BELT,REVERSER:2
- Mate:315: PLATE,BACK:1 ↔ PLATE,BELT,REVERSER:2
- Mate:316: WCP-2057:9 ↔ REV-21-1921:4
- Mate:317: REV-21-1921:3 ↔ WCP-2057:15
- Mate:318: WCP-2057:9 ↔ REV-21-1921:4
- Flush:66: REV-21-1921:3 ↔ REV-21-1921:4
- Mate:319: WCP-2057:12 ↔ WCP-0565:1
- Mate:320: WCP-2057:15 ↔ WCP-1420:8
- Mate:321: REV-21-1921:3 ↔ WCP-1420:8
- Insert:319: PLATE,BELT,REVERSER:2 ↔ WCP-2057:16
- Mate:322: WCP-1420:8 ↔ WCP-2057:16
- Flush:67: WCP-0565:1 ↔ WCP-1420:8
- Mate:323: PLATE,FRONT:1 ↔ KICKER_GEARBOX
- Mate:324: WCP-2057:13 ↔ WCP-1420:3
- Insert:320: PLATE,FRONT:1 ↔ WCP-2057:17
- Mate:325: PLATE,FRONT:1 ↔ KICKER_GEARBOX
- Mate:326: KICKER_GEARBOX ↔ WCP-1420:7
- Mate:327: PLATE,FRONT:1 ↔ 3DPRINT,KICKER,MOTOR,MOUNT:1
- Mate:328: PLATE,FRONT:1 ↔ 3DPRINT,KICKER,MOTOR,MOUNT:1
- Mate:329: PLATE,FRONT:1 ↔ 3DPRINT,KICKER,MOTOR,MOUNT:1
- Insert:321: 3DPRINT,NUT-BLOCK:1 ↔ PLATE,SHOOTER,MOUNT:1
- Mate:330: 3DPRINT,NUT-BLOCK:1 ↔ PLATE,SHOOTER,MOUNT:1
- Insert:322: PLATE,BACK:1 ↔ 3DPRINT,NUT-BLOCK:3
- Insert:323: PLATE,BACK:1 ↔ 3DPRINT,NUT-BLOCK:2
- Mate:331: PLATE,BACK:1 ↔ 3DPRINT,NUT-BLOCK:3
- Mate:332: PLATE,BACK:1 ↔ 3DPRINT,NUT-BLOCK:2
- Insert:324: PLATE,BACK:1 ↔ 3DPRINT,NUT-BLOCK:4
- Insert:325: PLATE,BACK:1 ↔ 3DPRINT,NUT-BLOCK:5
- Mate:333: PLATE,BACK:1 ↔ 3DPRINT,NUT-BLOCK:4
- Mate:334: PLATE,BACK:1 ↔ 3DPRINT,NUT-BLOCK:5
- Insert:326: PLATE,FRONT:1 ↔ 3DPRINT,NUT-BLOCK:6
- Mate:335: PLATE,FRONT:1 ↔ 3DPRINT,NUT-BLOCK:6
- Mate:336: PLATE,BACK:1 ↔ 3DPRINT,NUT-BLOCK:7
- Mate:337: PLATE,BACK:1 ↔ 3DPRINT,NUT-BLOCK:7
- Mate:338: PLATE,BACK:1 ↔ 3DPRINT,NUT-BLOCK:7
- Insert:327: PLATE,FRONT:1 ↔ 3DPRINT,NUT-BLOCK:8
- Insert:328: PLATE,BACK:1 ↔ 3DPRINT,NUT-BLOCK:13
- Insert:331: PLATE,FRONT:1 ↔ 3DPRINT,NUT-BLOCK:10
- Insert:332: PLATE,FRONT:1 ↔ 3DPRINT,NUT-BLOCK:9
- Mate:339: PLATE,FRONT:1 ↔ 3DPRINT,NUT-BLOCK:9
- Mate:340: PLATE,FRONT:1 ↔ 3DPRINT,NUT-BLOCK:10
- Mate:343: PLATE,FRONT:1 ↔ 3DPRINT,NUT-BLOCK:8
- Insert:333: PLATE,BACK:1 ↔ STOCK,REVERSER,STANDOFF:1
- Insert:334: PLATE,BACK:1 ↔ STOCK,REVERSER,STANDOFF:2
- Insert:335: PLATE,BACK:1 ↔ STOCK,REVERSER,STANDOFF:3
- Insert:336: PLATE,BACK:1 ↔ STOCK,REVERSER,STANDOFF:6
- Insert:337: PLATE,BACK:1 ↔ STOCK,REVERSER,STANDOFF:5
- Insert:338: PLATE,BACK:1 ↔ STOCK,REVERSER,STANDOFF:4
- Mate:344: PLATE,BACK:1 ↔ 3DPRINT,NUT-BLOCK:12
- Insert:339: PLATE,BACK:1 ↔ 3DPRINT,NUT-BLOCK:12
- Mate:345: PLATE,FRONT:1 ↔ 3DPRINT,NUT-BLOCK:11
- Insert:340: PLATE,FRONT:1 ↔ 3DPRINT,NUT-BLOCK:11
- Mate:346: 3DPRINT,BELT,GUARD:1 ↔ PLATE,SHOOTER,MOUNT:1
- Mate:347 (92.075 mm): PLATE,BACK:1 ↔ 3DPRINT,BELT,GUARD:1
- Mate:348 (26.3144 mm): 3DPRINT,BELT,GUARD:1 ↔ 3DPRINT,BELT,GUARD:2
- Mate:349: 3DPRINT,BELT,GUARD:2 ↔ PLATE,SHOOTER,MOUNT:1
- Flush:68: 3DPRINT,BELT,GUARD:1 ↔ 3DPRINT,BELT,GUARD:2
- [Mate] (26.3144 mm): 3DPRINT,BELT,GUARD:3 ↔ 3DPRINT,BELT,GUARD:4
- [Flush]: 3DPRINT,BELT,GUARD:3 ↔ 3DPRINT,BELT,GUARD:4
- Flush:70: 3DPRINT,BELT,GUARD:3 ↔ 3DPRINT,BELT,GUARD:4
- Flush:71: PLATE,BACK:1 ↔ 3DPRINT,BELT,GUARD:3
- Mate:351 (92.075 mm): PLATE,BACK:1 ↔ 3DPRINT,BELT,GUARD:3
- Flush:72: 3DPRINT,BELT,GUARD:1 ↔ 3DPRINT,BELT,GUARD:3
- Flush:73 (88.9 mm): PLATE,BACK:1 ↔ 3DPRINT,BELT,GUARD:4
- Mate:352 (1 mm): PLATE,BACK:1 ↔ 3DPRINT,BACK,RAIL:1
- Flush:74 (89.535 mm): PLATE,BACK:1 ↔ 3DPRINT,BACK,RAIL:1
- Flush:75 (88.9 mm): PLATE,BACK:1 ↔ 3DPRINT,BACK,RAIL:1
- Insert:341: PLATE,LEFT ↔ 3DPRINT,NUT-BLOCK:14
- Mate:353: PLATE,LEFT ↔ 3DPRINT,NUT-BLOCK:14
- Mate:354: PLATE,LEFT ↔ 3DPRINT,NUT-BLOCK:15
- Mate:355: PLATE,LEFT ↔ 3DPRINT,NUT-BLOCK:15
- Mate:356: PLATE,LEFT ↔ 3DPRINT,NUT-BLOCK:15
- Mate:357: PLATE,BACK:1 ↔ PLATE,RIGHT:1
- Mate:358: PLATE,RIGHT:1 ↔ PLATE,SHOOTER,MOUNT:1
- Flush:76: PLATE,BACK:1 ↔ PLATE,RIGHT:1
- Mate:359: 3DPRINT,VERTICAL,ROLLER,TOP,BEARING,BLOCK:1 ↔ WCP-1420:6
- Mate:360 (18.2563 mm): 3DPRINT,VERTICAL,ROLLER,TOP,BEARING,BLOCK:1 ↔ WCP-1420:6
- Mate:361: WCP-2057:14 ↔ STOCK,VERTICAL,HEX:1
- Flush:77: WCP-1420:6 ↔ STOCK,VERTICAL,HEX:1
- Insert:342: PLATE,BACK:1 ↔ 3DPRINT,NUT-BLOCK:17
- Mate:362: PLATE,BACK:1 ↔ 3DPRINT,NUT-BLOCK:17
- Insert:343: 3DPRINT,NUT-BLOCK:16 ↔ PLATE,SHOOTER,MOUNT:1
- Mate:363: 3DPRINT,NUT-BLOCK:16 ↔ PLATE,SHOOTER,MOUNT:1
- Mate:364: PLATE,RIGHT:1 ↔ 3DPRINT,LEFT,NUT-BLOCK:1
- Insert:344: PLATE,RIGHT:1 ↔ 3DPRINT,LEFT,NUT-BLOCK:1
## Named parameters: d747_d702 = 0 mm, d810_d807 = 26.3144 mm, d811_d809 = 0 mm
